# Autodesk Inventor assembly: Piston Assembly
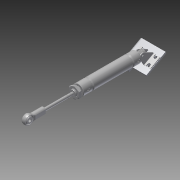
[picture p0: Inventor's stored thumbnail of the model, 180x180]
Saved by Autodesk Inventor 2014 (Build 180170000, 170)
## iProperties
Created: 2014-01-13
Part Number: Piston Assembly
Document SubType Name: Assembly
Designer: Michael
Mass: 287.707 g
Surface Area: 227.759 cm^2
Volume: 36.6506 cm^3
Density: 7.85 g/cm^3
Author: Michael
## Documents named in this file (5)
- C:\Users\Michael\Documents\GitHub\2014buildCAD\Collector\Piston Assembly.iam
- C:\Users\Michael\Documents\GitHub\2014buildCAD\Collector\Pneumatic Piston Front Connector (6498K592).ipt
- C:\Users\Michael\Documents\GitHub\2014buildCAD\Collector\Pneumatic Piston Pivot Mount (6498K710).ipt
- C:\Users\Michael\Documents\GitHub\2014buildCAD\Collector\Pneumatic Piston Back Flange (Custom).ipt
- C:\Users\Michael\Documents\GitHub\2014buildCAD\Collector\Pneumatic Piston 2 in Stroke 7-16 Bore (6498K604).ipt
## Components (4 placed, 4 different names)
1. Pneumatic Piston Front Connector (6498K592):1 — Angle:3, Mate:1, Mate:2
2. Pneumatic Piston Pivot Mount (6498K710):1 — Angle:3, Insert:2, Insert:3, Insert:4
3. Pneumatic Piston Back Flange (Custom):1 — Insert:2, Insert:3
4. Pneumatic Piston 2 in Stroke 7-16 Bore (6498K604):1 — Insert:4, Mate:1, Mate:2
## Relationships (6: Insert 3, Mate 2, Angle 1)
- Angle:3 (0 deg): Pneumatic Piston Front Connector (6498K592):1 ↔ Pneumatic Piston Pivot Mount (6498K710):1
- Insert:2: Pneumatic Piston Pivot Mount (6498K710):1 ↔ Pneumatic Piston Back Flange (Custom):1
- Insert:3: Pneumatic Piston Pivot Mount (6498K710):1 ↔ Pneumatic Piston Back Flange (Custom):1
- Insert:4: Pneumatic Piston Pivot Mount (6498K710):1 ↔ Pneumatic Piston 2 in Stroke 7-16 Bore (6498K604):1
- Mate:1: Pneumatic Piston Front Connector (6498K592):1 ↔ Pneumatic Piston 2 in Stroke 7-16 Bore (6498K604):1
- Mate:2 (-12.7 mm): Pneumatic Piston Front Connector (6498K592):1 ↔ Pneumatic Piston 2 in Stroke 7-16 Bore (6498K604):1
